# Autodesk Inventor assembly: testing2016
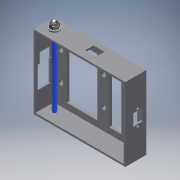
[picture p0: Inventor's stored thumbnail of the model, 180x180]
Saved by Autodesk Inventor 2017.2 (Build 212233000, 233)
## iProperties
Created: 2016-05-19
Part Number: testing2016
Document SubType Name: Assembly
Designer: steele
Author: steele
## Documents named in this file (3)
- D:\snobotics\CAD-Development\robSteele\testing2016.iam
- D:\snobotics\CAD-Development\robSteele\RaspberryPi\Pi Case Bottom V 01.ipt
- D:\snobotics\CAD-Development\robSteele\testing2016\Design Accelerator\Bolted Connection1.iam
## Components (2 placed, 2 different names)
1. Pi Case Bottom V 01:1 — Mate:1, Mate:2
2. Bolted Connection:1 [sub-assembly] — Mate:1, Mate:2
## Relationships (2: Mate 2)
- Mate:1: Pi Case Bottom V 01:1 ↔ Bolted Connection:1
- Mate:2: Pi Case Bottom V 01:1 ↔ Bolted Connection:1
